# Autodesk Inventor assembly: Nieuw zonnepaneel module
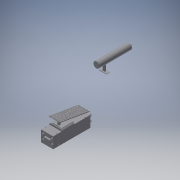
[picture p0: Inventor's stored thumbnail of the model, 180x180]
Saved by Autodesk Inventor 2018.3 (Build 223284000, 284)
## iProperties
Created: 2021-01-04
Part Number: Nieuw zonnepaneel module
Document SubType Name: Assembly
Designer: daanv
Author: daanv
## Documents named in this file (7)
- C:\Users\daanv\OneDrive\Documenten\Life\Avans Project RED\Token\Zonnepaneel\V6\Nieuw zonnepaneel module.iam
- C:\Users\daanv\OneDrive\Documenten\Life\Avans Project RED\Token\Zonnepaneel\V6\Bevestiging Token.ipt
- C:\Users\daanv\OneDrive\Documenten\Life\Avans Project RED\Token\Zonnepaneel\V6\updated token 18mm.ipt
- C:\Users\daanv\OneDrive\Documenten\Life\Avans Project RED\Token\Zonnepaneel\V6\Voorplaat.ipt
- C:\Users\daanv\OneDrive\Documenten\Life\Avans Project RED\Token\Zonnepaneel\V6\zij.ipt
- C:\Users\daanv\OneDrive\Documenten\Life\Avans Project RED\Token\Zonnepaneel\V6\Bevestiging Token Batterij.ipt
- C:\Users\daanv\OneDrive\Documenten\Life\Avans Project RED\Token\Zonnepaneel\V6\deksel token Nieuw bevestiging uitwendig.ipt
## Components (6 placed, 6 different names)
1. updated token 18mm:1 — Mate:1, Mate:3, Mate:4, Mate:6, Mate:7, Mate:8
2. Voorplaat:1 — Mate:1, Mate:3, Mate:4, Mate:9
3. zij:1 — Mate:6, Mate:7
4. Bevestiging Token:2 — Mate:10, Mate:11
5. Bevestiging Token Batterij:1
6. deksel token Nieuw bevestiging uitwendig:1 — Mate:8, Mate:9, Mate:10, Mate:11
## Relationships (9: Mate 9)
- Mate:1: updated token 18mm:1 ↔ Voorplaat:1
- Mate:3: updated token 18mm:1 ↔ Voorplaat:1
- Mate:4: updated token 18mm:1 ↔ Voorplaat:1
- Mate:6: updated token 18mm:1 ↔ zij:1
- Mate:7: updated token 18mm:1 ↔ zij:1
- Mate:8: updated token 18mm:1 ↔ deksel token Nieuw bevestiging uitwendig:1
- Mate:9: Voorplaat:1 ↔ deksel token Nieuw bevestiging uitwendig:1
- Mate:10: Bevestiging Token:2 ↔ deksel token Nieuw bevestiging uitwendig:1
- Mate:11: Bevestiging Token:2 ↔ deksel token Nieuw bevestiging uitwendig:1
